# Autodesk Inventor assembly: Connessione C
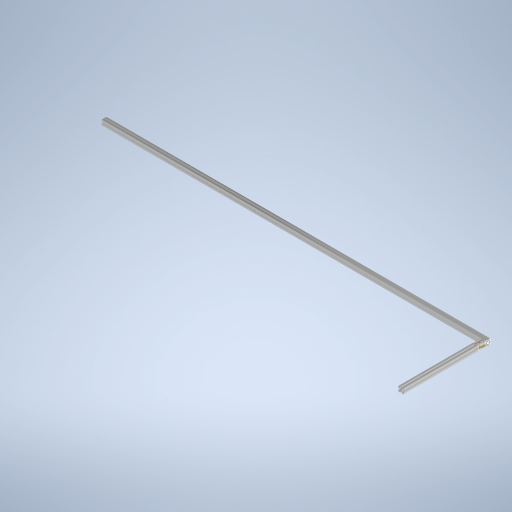
[picture p0: Inventor's stored thumbnail of the model, 512x512]
Saved by Autodesk Inventor 2023 (Build 270158000, 158)
## iProperties
Created: 2022-01-26
Part Number: Connessione C
Document SubType Name: Assembly
Designer: matte
Author: matte
## Documents named in this file (9)
- C:\Users\utente\OneDrive\Documenti\UniTN\I semestre\Connessione C.iam
- C:\Users\utente\OneDrive\Documenti\UniTN\I semestre\Mechanical Design\MDM-CyberOrto-CAD\Pezzi singoli\10-040.ipt
- C:\Users\utente\OneDrive\Documenti\UniTN\I semestre\Mechanical Design\MDM-CyberOrto-CAD\Parker components\05-Handles_Hinges\13-Pivot Joints\23-010.iam
- C:\Users\utente\OneDrive\Documenti\UniTN\I semestre\Mechanical Design\MDM-CyberOrto-CAD\Parker components\02-Fasteners\10-Standard T-Nuts\20-058.ipt
- C:\Users\utente\OneDrive\Documenti\UniTN\I semestre\Mechanical Design\MDM-CyberOrto-CAD\Parker components\02-Fasteners\16-Screws\01-Metric Screws\01-Button Head\24-116-8.ipt
- C:\Users\utente\OneDrive\Documenti\UniTN\I semestre\Mechanical Design\MDM-CyberOrto-CAD\Pezzi singoli\Supporto DX.ipt
- C:\Users\utente\OneDrive\Documenti\UniTN\I semestre\Mechanical Design\MDM-CyberOrto-CAD\Parker components\02-Fasteners\16-Screws\01-Metric Screws\01-Button Head\24-120-8.ipt
- C:\Users\utente\OneDrive\Documenti\UniTN\I semestre\Mechanical Design\MDM-CyberOrto-CAD\Pezzi singoli\13-106_f.ipt
- C:\Users\utente\OneDrive\Documenti\UniTN\I semestre\Mechanical Design\MDM-CyberOrto-CAD\Pezzi singoli\13-513.ipt
## Components (10 placed, 8 different names)
1. 23-010:1 [sub-assembly]
2. 20-058:1
3. 24-116-8:1
4. Supporto DX:1
5. 24-120-8:1
6. 13-106_f:1
7. 13-106_f:2
8. 13-513:1
9. 13-513:2
10. 10-040:2
## Relationships (23: Mate 14, Flush 8, Angle 1)
- [Mate]: 23-010:1 ↔ 10-040:2
- [Flush]: 23-010:1 ↔ 10-040:2
- [Flush]: 23-010:1 ↔ 10-040:2
- [Mate]: 20-058:1 ↔ 10-040:2
- [Angle] (0 deg): 20-058:1 ↔ 10-040:2
- [Mate]: 20-058:1 ↔ 24-116-8:1
- [Mate]: 23-010:1 ↔ 24-116-8:1
- [Mate]: 23-010:1 ↔ 24-116-8:1
- [Mate]: 23-010:1 ↔ Supporto DX:1
- [Flush]: 23-010:1 ↔ Supporto DX:1
- [Flush]: 23-010:1 ↔ Supporto DX:1
- [Mate]: 23-010:1 ↔ 24-120-8:1
- [Mate]: 23-010:1 ↔ 24-120-8:1
- [Flush]: 13-106_f:2 ↔ 10-040:2
- [Mate]: 13-106_f:2 ↔ 10-040:2
- [Mate]: 13-106_f:2 ↔ 10-040:2
- [Flush]: 13-106_f:1 ↔ 10-040:2
- [Mate]: 13-106_f:1 ↔ 10-040:2
- [Mate]: 13-106_f:1 ↔ 10-040:2
- [Flush]: 13-513:1 ↔ 10-040:2
- [Flush]: 13-513:2 ↔ 10-040:2
- [Mate]: 13-106_f:2 ↔ 13-513:2
- [Mate]: 13-106_f:1 ↔ 13-513:1
## Named parameters: d39_d48 = 0 mm, d40_d49 = 0 mm, d41_d50 = 0 mm, d42_d51 = 0 mm
